# Autodesk Inventor assembly: top_flange
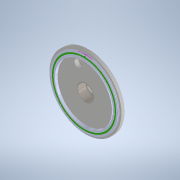
[picture p0: Inventor's stored thumbnail of the model, 180x180]
Saved by Autodesk Inventor 2021 (Build 250183000, 183)
## iProperties
Created: 2024-02-13
Part Number: top_flange
Document SubType Name: Assembly
Designer: Sebastián
Author: Sebastián
## Documents named in this file (7)
- C:\Users\Sebastián\Documents\Inventor\PLD SAP\top_flange.iam
- C:\Users\Sebastián\Documents\Inventor\PLD SAP\top_flange.ipt
- C:\Users\Sebastián\Documents\Inventor\PLD_Chamber\Hositrad_KF40-44.5-30.ipt
- C:\Users\Sebastián\Documents\Inventor\PLD_Chamber\Hositrad_KF16-20-20.ipt
- C:\Users\Sebastián\Documents\Inventor\PLD SAP\Hositrad_KF40B.ipt
- C:\Users\Sebastián\Documents\Inventor\PLD SAP\top_window.ipt
- C:\Users\Sebastián\Documents\Inventor\PLD SAP\Hositrad_ISO160AV.ipt
## Components (6 placed, 6 different names)
1. top_flange:1 — Cylindrical:3, Cylindrical:4, Rotational:7, Flush:1, Flush:2
2. Hositrad_KF40-44.5-30:1 — Cylindrical:3, Cylindrical:7, Flush:1
3. Hositrad_KF16-20-20:1 — Cylindrical:4, Flush:2
4. Hositrad_KF40B:1 — Rotational:5, Cylindrical:7
5. top_window:1 — Rotational:5
6. Hositrad_ISO160AV:1 — Rotational:7
## Relationships (7: CylindricalJoint 3, RevoluteJoint 2, Flush 2)
- Cylindrical:3: top_flange:1 ↔ Hositrad_KF40-44.5-30:1
- Cylindrical:4: top_flange:1 ↔ Hositrad_KF16-20-20:1
- Rotational:5 [RevoluteJoint]: Hositrad_KF40B:1 ↔ top_window:1
- Cylindrical:7: Hositrad_KF40-44.5-30:1 ↔ Hositrad_KF40B:1
- Rotational:7 [RevoluteJoint]: top_flange:1 ↔ Hositrad_ISO160AV:1
- Flush:1 (7.5 mm): top_flange:1 ↔ Hositrad_KF40-44.5-30:1
- Flush:2 (-18 mm): top_flange:1 ↔ Hositrad_KF16-20-20:1
